# Autodesk Inventor assembly: bowl_assy
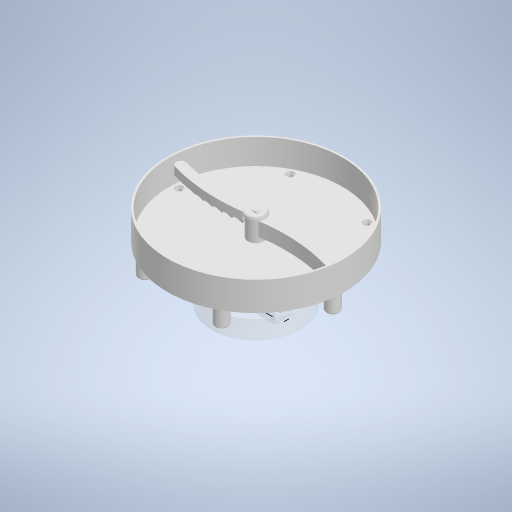
[picture p0: Inventor's stored thumbnail of the model, 512x512]
Saved by Autodesk Inventor 2023 (Build 270158000, 158)
## iProperties
Created: 2025-12-21
Part Number: bowl_assy
Document SubType Name: Assembly
Designer: Justin Pascual
Author: Justin Pascual
## Documents named in this file (13)
- C:\Users\Justin Pascual\Documents\GitHub\calming-sand-disk\bowl_assy.iam
- C:\Users\Justin Pascual\Documents\GitHub\calming-sand-disk\bowl.ipt
- C:\Users\Justin Pascual\Documents\GitHub\calming-sand-disk\legs.ipt
- C:\Users\Justin Pascual\Documents\GitHub\calming-sand-disk\hub.ipt
- C:\Users\Justin Pascual\Documents\GitHub\calming-sand-disk\rake_arm.ipt
- C:\Users\Justin Pascual\Documents\GitHub\calming-sand-disk\blade_arm.ipt
- C:\Users\Justin Pascual\Documents\GitHub\calming-sand-disk\cap.ipt
- C:\Users\Justin Pascual\Documents\GitHub\calming-sand-disk\bottom_thread.ipt
- C:\Users\Justin Pascual\Documents\GitHub\calming-sand-disk\bottom_basket.ipt
- C:\Users\Justin Pascual\Documents\GitHub\calming-sand-disk\bevel_gear_large.ipt
- C:\Users\Justin Pascual\Documents\GitHub\calming-sand-disk\bevel_gear_small.ipt
- C:\Users\Justin Pascual\Documents\GitHub\distillery-space-spinner\motor.ipt
- C:\Users\Justin Pascual\Documents\GitHub\calming-sand-disk\bevel_gears.iam
## Components (17 placed, 12 different names)
1. bowl:1 — Mate:1, Mate:2, Mate:3, Mate:4, Mate:5, Mate:6, Mate:7, Mate:8, Mate:9, Mate:10, Mate:11, Mate:12, Mate:13, Mate:14, Mate:25, Mate:26, Mate:27, Mate:28, Angle:2, Mate:30, Mate:32, Angle:4, Mate:34
2. legs:1 — Mate:1, Mate:7
3. legs:2 — Mate:2, Mate:9
4. legs:3 — Mate:3, Mate:10
5. legs:4 — Mate:4, Mate:11
6. legs:5 — Mate:6, Mate:8
7. legs:6 — Mate:5, Mate:12
8. hub:1 — Mate:13, Mate:14, Mate:18, Mate:19, Mate:20, Mate:21, Mate:22, Mate:23, Mate:24
9. rake_arm:1 — Mate:18, Mate:19, Mate:20
10. blade_arm:1 — Mate:21, Mate:22
11. cap:1 — Mate:23, Mate:24
12. bottom_thread:1 — Mate:25, Mate:26
13. bottom_basket:1 — Mate:27, Mate:28, Angle:3
14. Bevel Gear2:1 — Angle:2, Mate:29, Mate:30, Mate:32
15. Bevel Gear1:1 — Angle:1, Mate:29, Mate:31, Flush:1
16. motor:1 — Mate:31, Flush:1, Angle:3, Mate:33
17. bevel_gears:1 [sub-assembly] — Mate:33, Angle:4, Mate:34
## Relationships (36: Mate 31, Angle 4, Flush 1)
- Mate:1: bowl:1 ↔ legs:1
- Mate:2: bowl:1 ↔ legs:2
- Mate:3: bowl:1 ↔ legs:3
- Mate:4: bowl:1 ↔ legs:4
- Mate:5: bowl:1 ↔ legs:6
- Mate:6: bowl:1 ↔ legs:5
- Mate:7: bowl:1 ↔ legs:1
- Mate:8: bowl:1 ↔ legs:5
- Mate:9: bowl:1 ↔ legs:2
- Mate:10: bowl:1 ↔ legs:3
- Mate:11: bowl:1 ↔ legs:4
- Mate:12: bowl:1 ↔ legs:6
- Mate:13: bowl:1 ↔ hub:1
- Mate:14: bowl:1 ↔ hub:1
- Mate:18: hub:1 ↔ rake_arm:1
- Mate:19: hub:1 ↔ rake_arm:1
- Mate:20: hub:1 ↔ rake_arm:1
- Mate:21: hub:1 ↔ blade_arm:1
- Mate:22: hub:1 ↔ blade_arm:1
- Mate:23: hub:1 ↔ cap:1
- Mate:24: hub:1 ↔ cap:1
- Mate:25: bowl:1 ↔ bottom_thread:1
- Mate:26: bowl:1 ↔ bottom_thread:1
- Mate:27: bowl:1 ↔ bottom_basket:1
- Mate:28: bowl:1 ↔ bottom_basket:1
- Angle:1 (0 deg): Bevel Gear1:1
- Angle:2 (0 deg): bowl:1 ↔ Bevel Gear2:1
- Mate:29: Bevel Gear2:1 ↔ Bevel Gear1:1
- Mate:30 (2.54 mm): bowl:1 ↔ Bevel Gear2:1
- Mate:31: Bevel Gear1:1 ↔ motor:1
- Mate:32: bowl:1 ↔ Bevel Gear2:1
- Flush:1: Bevel Gear1:1 ↔ motor:1
- Angle:3 (0 deg): bottom_basket:1 ↔ motor:1
- Mate:33: motor:1 ↔ bevel_gears:1
- Angle:4 (180 deg): bowl:1 ↔ bevel_gears:1
- Mate:34: bowl:1 ↔ bevel_gears:1
